# Autodesk Inventor assembly: Assembly1
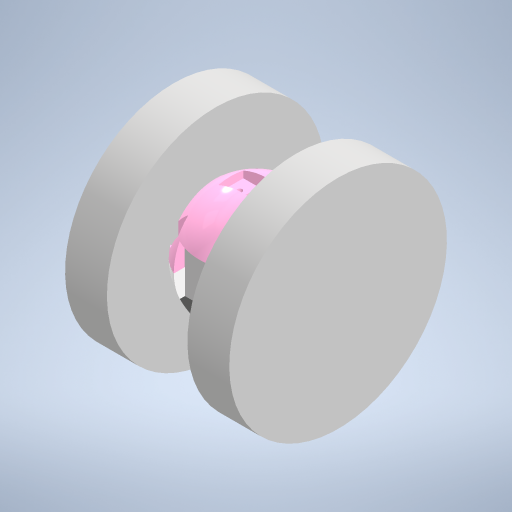
[picture p0: Inventor's stored thumbnail of the model, 512x512]
Saved by Autodesk Inventor 2023 (Build 270158000, 158)
## iProperties
Created: 2022-10-24
Part Number: Assembly1
Document SubType Name: Assembly
Designer: ellie
Author: ellie
## Documents named in this file (10)
- C:\Users\RM206user\Desktop\cansat\tanekonsat2022_runback\machinary\assenbly\Assembly1.iam
- C:\Users\RM206user\Desktop\cansat\tanekonsat2022_runback\machinary\body\body back\back moter middle tire ver\back moter middle tire lemon shape.ipt
- C:\Users\RM206user\Desktop\cansat\tanekonsat2022_runback\machinary\body\body back\back for main connection\body back for main 3.ipt
- C:\Users\RM206user\Desktop\cansat\tanekonsat2022_runback\machinary\parts\almi1.ipt
- C:\Users\RM206user\Desktop\cansat\tanekonsat2022_runback\machinary\parts\GNSS1.ipt
- C:\Users\RM206user\Desktop\cansat\tanekonsat2022_runback\machinary\parts\mein1.ipt
- C:\Users\RM206user\Desktop\cansat\tanekonsat2022_runback\machinary\parts\almi2.ipt
- C:\Users\RM206user\Desktop\cansat\tanekonsat2022_runback\machinary\body\body front\front moter middle basic\body front moter middle lemon shape.ipt
- C:\Users\RM206user\Desktop\cansat\tanekonsat2022_runback\machinary\parts\bush.ipt
- C:\Users\RM206user\Desktop\cansat\tanekonsat2022_runback\machinary\parts\tire\tire base\tire 130 25.ipt
## Components (14 placed, 9 different names)
1. body moter middle:1 — メイト:1, メイト:2, メイト:3, メイト:4, メイト:5, メイト:6
2. body moter middle:2 — メイト:1, メイト:2, メイト:3
3. body back:3 — メイト:4, メイト:5, メイト:6
4. almi1:1 — メイト:32, メイト:33, メイト:34
5. GNSS1:1 — メイト:35, メイト:36, メイト:37
6. mein1:1 — メイト:29, メイト:30, メイト:31
7. almi2:1 — メイト:26, メイト:27, メイト:28
8. body moter middle:4 — メイト:18, メイト:19, メイト:20, メイト:27, メイト:28, メイト:30, メイト:31, メイト:33, メイト:34, メイト:36, メイト:37, メイト:38, メイト:39, メイト:40, メイト:41, メイト:44
9. body back:5 — メイト:18, メイト:19, メイト:20, メイト:26, メイト:29, メイト:32, メイト:35
10. base front:1 — メイト:38, メイト:39, メイト:40, メイト:42, メイト:43, メイト:48
11. bush:1 — メイト:41, メイト:42, メイト:45, メイト:46
12. bush:2 — メイト:43, メイト:44, メイト:47
13. tire 130 25:1 — メイト:47, メイト:48
14. tire 130 25:2 — メイト:45, メイト:46
## Relationships (32: Mate 32)
- メイト:1 [Mate]: body moter middle:1 ↔ body moter middle:2
- メイト:2 [Mate]: body moter middle:1 ↔ body moter middle:2
- メイト:3 [Mate]: body moter middle:1 ↔ body moter middle:2
- メイト:4 [Mate]: body moter middle:1 ↔ body back:3
- メイト:5 [Mate]: body moter middle:1 ↔ body back:3
- メイト:6 [Mate]: body moter middle:1 ↔ body back:3
- メイト:18 [Mate]: body moter middle:4 ↔ body back:5
- メイト:19 [Mate]: body moter middle:4 ↔ body back:5
- メイト:20 [Mate]: body moter middle:4 ↔ body back:5
- メイト:26 [Mate]: almi2:1 ↔ body back:5
- メイト:27 [Mate]: almi2:1 ↔ body moter middle:4
- メイト:28 [Mate]: almi2:1 ↔ body moter middle:4
- メイト:29 [Mate]: mein1:1 ↔ body back:5
- メイト:30 [Mate]: mein1:1 ↔ body moter middle:4
- メイト:31 [Mate]: mein1:1 ↔ body moter middle:4
- メイト:32 [Mate]: almi1:1 ↔ body back:5
- メイト:33 [Mate]: almi1:1 ↔ body moter middle:4
- メイト:34 [Mate]: almi1:1 ↔ body moter middle:4
- メイト:35 [Mate]: GNSS1:1 ↔ body back:5
- メイト:36 [Mate]: GNSS1:1 ↔ body moter middle:4
- メイト:37 [Mate]: GNSS1:1 ↔ body moter middle:4
- メイト:38 [Mate]: body moter middle:4 ↔ base front:1
- メイト:39 [Mate]: body moter middle:4 ↔ base front:1
- メイト:40 [Mate]: body moter middle:4 ↔ base front:1
- メイト:41 [Mate]: body moter middle:4 ↔ bush:1
- メイト:42 [Mate]: base front:1 ↔ bush:1
- メイト:43 [Mate]: base front:1 ↔ bush:2
- メイト:44 [Mate]: body moter middle:4 ↔ bush:2
- メイト:45 [Mate] (-20 mm): bush:1 ↔ tire 130 25:2
- メイト:46 [Mate]: bush:1 ↔ tire 130 25:2
- メイト:47 [Mate] (-20 mm): bush:2 ↔ tire 130 25:1
- メイト:48 [Mate]: base front:1 ↔ tire 130 25:1
